# Autodesk Inventor assembly: Koruza U-peofil
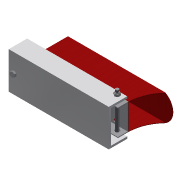
[picture p0: Inventor's stored thumbnail of the model, 180x180]
Saved by Autodesk Inventor 2015 (Build 190159000, 159)
## iProperties
Created: 2015-01-09
Part Number: Koruza U-peofil
Document SubType Name: Assembly
Designer: Michal
Author: Michal
## Documents named in this file (7)
- C:\Users\Michal\Desktop\Michal\Prace\koruza\Koruza U-peofil.iam
- C:\Users\Michal\Desktop\Michal\Prace\koruza\Case.ipt
- C:\Users\Michal\Desktop\Michal\Prace\koruza\U-profil 100x40 - pod case.ipt
- C:\Users\Michal\Desktop\Michal\Prace\koruza\U profil 140x70 základní.ipt
- C:\Users\Michal\Desktop\Michal\Prace\koruza\Šrouv M12x60.ipt
- C:\Users\Michal\Desktop\Michal\Prace\koruza\ANSI B18.16.3M - Property Class 5 and 10 - Metric M12 x 1.75 Typ kovu.ipt
- C:\Users\Michal\Desktop\Michal\Prace\koruza\ISO 4035 - M12ISO.ipt
## Components (11 placed, 6 different names)
1. Case:1 — Proti sobě:1, Stejný směr:1, Stejný směr:2
2. U-profil 100x40 - pod case:1 — Proti sobě:1, Stejný směr:1, Stejný směr:2, Proti sobě:2, Stejný směr:3, Proti sobě:3, Proti sobě:9, Proti sobě:11, Proti sobě:15, Proti sobě:17
3. U profil 140x70 základní:1 — Proti sobě:2, Stejný směr:3, Proti sobě:3, Proti sobě:4, Proti sobě:5, Proti sobě:7, Proti sobě:12, Proti sobě:13, Proti sobě:18
4. Šrouv M12x60:1 — Proti sobě:4, Proti sobě:5, Proti sobě:6, Proti sobě:8, Proti sobě:10
5. ANSI B18.16.3M - Property Class 5 and 10 - Metric M12 x 1.75 Typ kovu:1 — Proti sobě:6, Proti sobě:7
6. ISO 4035 - M12ISO:1 — Proti sobě:8, Proti sobě:9
7. ISO 4035 - M12ISO:2 — Proti sobě:10, Proti sobě:11
8. Šrouv M12x60:2 — Proti sobě:12, Proti sobě:13, Proti sobě:14, Proti sobě:16, Proti sobě:19
9. ANSI B18.16.3M - Property Class 5 and 10 - Metric M12 x 1.75 Typ kovu:2 — Proti sobě:18, Proti sobě:19
10. ISO 4035 - M12ISO:3 — Proti sobě:16, Proti sobě:17
11. ISO 4035 - M12ISO:4 — Proti sobě:14, Proti sobě:15
## Relationships (22: Mate 19, Flush 3)
- Proti sobě:1 [Mate]: Case:1 ↔ U-profil 100x40 - pod case:1
- Stejný směr:1 [Flush]: Case:1 ↔ U-profil 100x40 - pod case:1
- Stejný směr:2 [Flush] (-50 mm): Case:1 ↔ U-profil 100x40 - pod case:1
- Proti sobě:2 [Mate]: U-profil 100x40 - pod case:1 ↔ U profil 140x70 základní:1
- Stejný směr:3 [Flush] (15 mm): U-profil 100x40 - pod case:1 ↔ U profil 140x70 základní:1
- Proti sobě:3 [Mate]: U-profil 100x40 - pod case:1 ↔ U profil 140x70 základní:1
- Proti sobě:4 [Mate]: U profil 140x70 základní:1 ↔ Šrouv M12x60:1
- Proti sobě:5 [Mate]: U profil 140x70 základní:1 ↔ Šrouv M12x60:1
- Proti sobě:6 [Mate]: Šrouv M12x60:1 ↔ ANSI B18.16.3M - Property Class 5 and 10 - Metric M12 x 1.75 Typ kovu:1
- Proti sobě:7 [Mate]: U profil 140x70 základní:1 ↔ ANSI B18.16.3M - Property Class 5 and 10 - Metric M12 x 1.75 Typ kovu:1
- Proti sobě:8 [Mate]: Šrouv M12x60:1 ↔ ISO 4035 - M12ISO:1
- Proti sobě:9 [Mate]: U-profil 100x40 - pod case:1 ↔ ISO 4035 - M12ISO:1
- Proti sobě:10 [Mate]: Šrouv M12x60:1 ↔ ISO 4035 - M12ISO:2
- Proti sobě:11 [Mate]: U-profil 100x40 - pod case:1 ↔ ISO 4035 - M12ISO:2
- Proti sobě:12 [Mate]: U profil 140x70 základní:1 ↔ Šrouv M12x60:2
- Proti sobě:13 [Mate]: U profil 140x70 základní:1 ↔ Šrouv M12x60:2
- Proti sobě:14 [Mate]: Šrouv M12x60:2 ↔ ISO 4035 - M12ISO:4
- Proti sobě:15 [Mate]: U-profil 100x40 - pod case:1 ↔ ISO 4035 - M12ISO:4
- Proti sobě:16 [Mate]: Šrouv M12x60:2 ↔ ISO 4035 - M12ISO:3
- Proti sobě:17 [Mate]: U-profil 100x40 - pod case:1 ↔ ISO 4035 - M12ISO:3
- Proti sobě:18 [Mate]: U profil 140x70 základní:1 ↔ ANSI B18.16.3M - Property Class 5 and 10 - Metric M12 x 1.75 Typ kovu:2
- Proti sobě:19 [Mate]: Šrouv M12x60:2 ↔ ANSI B18.16.3M - Property Class 5 and 10 - Metric M12 x 1.75 Typ kovu:2
